# Autodesk Inventor assembly: Camera OV7670
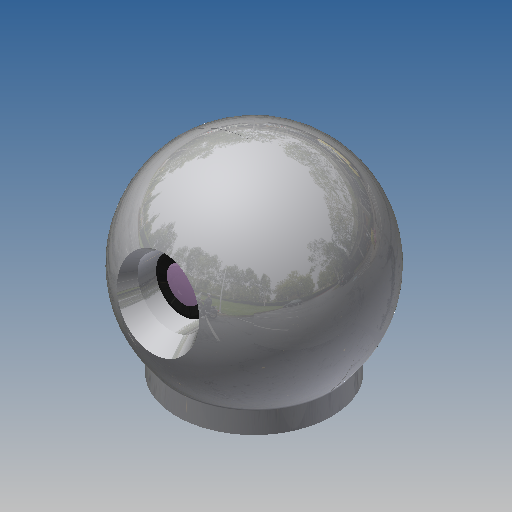
[picture p0: Inventor's stored thumbnail of the model, 512x512]
Saved by Autodesk Inventor 2020 (Build 240168000, 168)
## iProperties
Created: 2019-07-17
Part Number: Camera OV7670
Description: STEP AP214
Document SubType Name: Assembly
Designer: User
Sending System: SolidWorks 2016
Preprocessor: SwSTEP 2.0
Title: Camera OV7670.STEP
Author: VR
Revision Number: ANY
## Documents named in this file (13)
- F:\GrabCAD\Robot\Camera OV7670.iam
- F:\GrabCAD\Robot\PcbForCamera.ipt
- F:\GrabCAD\Robot\CameraLens.ipt
- F:\GrabCAD\Robot\pan head cross recess screw_iso_ISO 7045 - M1.6 x 6 - Z - 6N.ipt
- F:\GrabCAD\Robot\PLS (DS1021-2xN)_DS1021-2x9.ipt
- F:\GrabCAD\Robot\CAP 1206_Џ® г¬®«з ­Ёо.ipt
- F:\GrabCAD\Robot\CAP 0603_Џ® г¬®«з ­Ёо.ipt
- F:\GrabCAD\Robot\Stackpole CSR0402 Res_Џ® г¬®«з ­Ёо.ipt
- F:\GrabCAD\Robot\SC-70-5_Џ® г¬®«з ­Ёо.ipt
- F:\GrabCAD\Robot\CAMERA_COVER_1.ipt
- F:\GrabCAD\Robot\CAMERA_COVER_2.ipt
- F:\GrabCAD\Robot\AS 1427 - M3 x 8(5) II.ipt
- F:\GrabCAD\Robot\Деталь4.ipt
## Components (29 placed, 25 different names)
1. PcbForCamera_1 — Допуск симметричности:1, Заподлицо:4, Заподлицо:5, Заподлицо:6, Совмещение:5
2. CameraLens_2 — Допуск симметричности:1
3. pan head cross recess screw_iso_ISO 7045 - M1.6 x 6 - Z - 6N_3
4. pan head cross recess screw_iso_ISO 7045 - M1.6 x 6 - Z - 6N_4
5. PLS (DS1021-2xN)_DS1021-2x9_5
6. CAP 1206_Џ® г¬®«з ­Ёо_6
7. CAP 1206_Џ® г¬®«з ­Ёо_7
8. CAP 1206_Џ® г¬®«з ­Ёо_8
9. CAP 1206_Џ® г¬®«з ­Ёо_9
10. CAP 1206_Џ® г¬®«з ­Ёо_10
11. CAP 0603_Џ® г¬®«з ­Ёо_11
12. CAP 0603_Џ® г¬®«з ­Ёо_12
13. CAP 0603_Џ® г¬®«з ­Ёо_13
14. CAP 0603_Џ® г¬®«з ­Ёо_14
15. CAP 0603_Џ® г¬®«з ­Ёо_15
16. CAP 0603_Џ® г¬®«з ­Ёо_16
17. Stackpole CSR0402 Res_Џ® г¬®«з ­Ёо_17
18. Stackpole CSR0402 Res_Џ® г¬®«з ­Ёо_18
19. SC-70-5_Џ® г¬®«з ­Ёо_19
20. SC-70-5_Џ® г¬®«з ­Ёо_20
21. Stackpole CSR0402 Res_Џ® г¬®«з ­Ёо_21
22. CAMERA_COVER_1:1 — Заподлицо:1, Заподлицо:2, Заподлицо:3, Заподлицо:4, Заподлицо:5, Заподлицо:6, Заподлицо:7, Заподлицо:8, Совмещение:1, Совмещение:2, Совмещение:3, Совмещение:4
23. CAMERA_COVER_2:1 — Заподлицо:7, Заподлицо:8, Заподлицо:12, Заподлицо:13, Совмещение:6, Совмещение:7
24. AS 1427 H - метрическая M3 x 8:1 — Заподлицо:10, Заподлицо:11, Совмещение:1, Совмещение:5
25. AS 1427 H - метрическая M3 x 8:2 — Заподлицо:11, Совмещение:2
26. AS 1427 H - метрическая M3 x 8:3 — Заподлицо:9, Совмещение:4
27. AS 1427 H - метрическая M3 x 8:4 — Заподлицо:9, Заподлицо:10, Совмещение:3
28. Деталь4:1 — Заподлицо:12, Заподлицо:13, Заподлицо:14
29. Деталь4:2 — Заподлицо:14, Совмещение:6, Совмещение:7
## Relationships (22: Flush 14, Mate 7, Symmetry 1)
- Допуск симметричности:1 [Symmetry]: PcbForCamera_1 ↔ CameraLens_2
- Заподлицо:1 [Flush]: CAMERA_COVER_1:1
- Заподлицо:2 [Flush]: CAMERA_COVER_1:1
- Заподлицо:3 [Flush]: CAMERA_COVER_1:1
- Заподлицо:4 [Flush]: PcbForCamera_1 ↔ CAMERA_COVER_1:1
- Заподлицо:5 [Flush]: PcbForCamera_1 ↔ CAMERA_COVER_1:1
- Заподлицо:6 [Flush]: PcbForCamera_1 ↔ CAMERA_COVER_1:1
- Заподлицо:7 [Flush]: CAMERA_COVER_1:1 ↔ CAMERA_COVER_2:1
- Заподлицо:8 [Flush]: CAMERA_COVER_1:1 ↔ CAMERA_COVER_2:1
- Заподлицо:9 [Flush]: AS 1427 H - метрическая M3 x 8:3 ↔ AS 1427 H - метрическая M3 x 8:4
- Заподлицо:10 [Flush]: AS 1427 H - метрическая M3 x 8:1 ↔ AS 1427 H - метрическая M3 x 8:4
- Заподлицо:11 [Flush]: AS 1427 H - метрическая M3 x 8:1 ↔ AS 1427 H - метрическая M3 x 8:2
- Совмещение:1 [Mate]: CAMERA_COVER_1:1 ↔ AS 1427 H - метрическая M3 x 8:1
- Совмещение:2 [Mate]: CAMERA_COVER_1:1 ↔ AS 1427 H - метрическая M3 x 8:2
- Совмещение:3 [Mate]: CAMERA_COVER_1:1 ↔ AS 1427 H - метрическая M3 x 8:4
- Совмещение:4 [Mate]: CAMERA_COVER_1:1 ↔ AS 1427 H - метрическая M3 x 8:3
- Совмещение:5 [Mate]: PcbForCamera_1 ↔ AS 1427 H - метрическая M3 x 8:1
- Заподлицо:12 [Flush]: CAMERA_COVER_2:1 ↔ Деталь4:1
- Заподлицо:13 [Flush]: CAMERA_COVER_2:1 ↔ Деталь4:1
- Заподлицо:14 [Flush]: Деталь4:1 ↔ Деталь4:2
- Совмещение:6 [Mate] (0.1 mm): CAMERA_COVER_2:1 ↔ Деталь4:2
- Совмещение:7 [Mate] (0.1 mm): CAMERA_COVER_2:1 ↔ Деталь4:2
